# Autodesk Inventor assembly: motor assembly
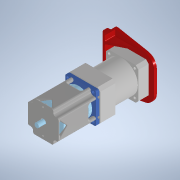
[picture p0: Inventor's stored thumbnail of the model, 180x180]
Saved by Autodesk Inventor 2021.3 (Build 253353000, 353)
## iProperties
Created: 2021-10-06
Part Number: motor assembly
Document SubType Name: Assembly
Designer: nxf77172
Mass: 1035.43 g
Surface Area: 842.407 cm^2
Volume: 462.38 cm^3
Density: 2.23934 g/cm^3
Author: nxf77172
## Documents named in this file (4)
- C:\Users\nxf77172\Desktop\mechanical_cleaned\custom_parts\drivetrain\motor assembly.iam
- C:\Users\nxf77172\Desktop\mechanical_cleaned\custom_parts\drivetrain\Gearbox.ipt
- C:\Users\nxf77172\Desktop\mechanical_cleaned\custom_parts\drivetrain\Motor - nat. cooling.ipt
- C:\Users\nxf77172\Desktop\mechanical_cleaned\custom_parts\drivetrain\gearbox_mounting_plate.ipt
## Components (3 placed, 3 different names)
1. Gearbox:1 — Mate:1, Mate:2, Mate:3, Flush:1, Angle:1, Angle:2, Flush:2, Flush:3
2. Motor - nat. cooling:1 — Mate:1, Mate:2, Angle:2
3. gearbox_mounting_plate:1 — Flush:2, Flush:3
## Relationships (8: Mate 3, Flush 3, Angle 2)
- Mate:1: Gearbox:1 ↔ Motor - nat. cooling:1
- Mate:2: Gearbox:1 ↔ Motor - nat. cooling:1
- Mate:3: Gearbox:1
- Flush:1: Gearbox:1
- Angle:1 (0 deg): Gearbox:1
- Angle:2 (0 deg): Gearbox:1 ↔ Motor - nat. cooling:1
- Flush:2: Gearbox:1 ↔ gearbox_mounting_plate:1
- Flush:3: Gearbox:1 ↔ gearbox_mounting_plate:1
